# Autodesk Inventor assembly: Assembly_Mão
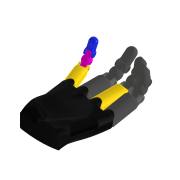
[picture p0: Inventor's stored thumbnail of the model, 180x180]
Saved by Autodesk Inventor 2020 (Build 240168000, 168)
## iProperties
Created: 2021-03-31
Part Number: Assembly_Mão
Document SubType Name: Assembly
Designer: deox
Author: deox
## Documents named in this file (17)
- C:\Users\deox\Desktop\TCC\Inventor Files\Dedo Kick\Assembly_Mão.iam
- C:\Users\deox\Desktop\TCC\Inventor Files\Dedo Kick\Base da Mão.ipt
- C:\Users\deox\Desktop\TCC\Inventor Files\Dedo Kick\Socket_Minimo.ipt
- C:\Users\deox\Desktop\TCC\Inventor Files\Dedo Kick\Cross_Minimo.ipt
- C:\Users\deox\Desktop\TCC\Inventor Files\Dedo Kick\Cross_Normal.ipt
- C:\Users\deox\Desktop\TCC\Inventor Files\Dedo Kick\Socket.ipt
- C:\Users\deox\Desktop\TCC\Inventor Files\Dedo Kick\Socket_Medio.ipt
- C:\Users\deox\Desktop\TCC\Inventor Files\Dedo Kick\Base_Minimo.ipt
- C:\Users\deox\Desktop\TCC\Inventor Files\Dedo Kick\Base.ipt
- C:\Users\deox\Desktop\TCC\Inventor Files\Dedo Kick\Middle_Minimo.ipt
- C:\Users\deox\Desktop\TCC\Inventor Files\Dedo Kick\Middle.ipt
- C:\Users\deox\Desktop\TCC\Inventor Files\Dedo Kick\ShameHider_Minimo.ipt
- C:\Users\deox\Desktop\TCC\Inventor Files\Dedo Kick\ShameHider.ipt
- C:\Users\deox\Desktop\TCC\Inventor Files\Dedo Kick\Tip_Minimo_ScaledDown.ipt
- C:\Users\deox\Desktop\TCC\Inventor Files\Dedo Kick\Tip.ipt
- C:\Users\deox\Desktop\TCC\Inventor Files\Dedo Kick\TipTip_Minimo.ipt
- C:\Users\deox\Desktop\TCC\Inventor Files\Dedo Kick\TipTip.ipt
## Components (29 placed, 16 different names)
1. Base da Mão:1 — Mate:3, Mate:4, Angle:1, Mate:7, Mate:8, Angle:2, Mate:11, Mate:12, Angle:3, Mate:15, Mate:16, Angle:4
2. Socket_Minimo:1 — Mate:1, Mate:2, Angle:1, Mate:17, Mate:18, Angle:5
3. Cross_Minimo:1 — Mate:1, Mate:2, Mate:3, Mate:4
4. Cross_Normal:1 — Mate:13, Mate:14, Mate:15, Mate:16
5. Cross_Normal:2 — Mate:9, Mate:10, Mate:11, Mate:12
6. Cross_Normal:3 — Mate:5, Mate:6, Mate:7, Mate:8
7. Socket:1 — Mate:13, Mate:14, Angle:4, Mate:23, Mate:24, Angle:8
8. Socket:2 — Mate:9, Mate:10, Angle:3, Mate:19, Mate:20, Angle:6
9. Socket_Medio:1 — Mate:5, Mate:6, Angle:2, Mate:21, Mate:22, Angle:7
10. Base_Minimo:1 — Mate:17, Mate:18, Angle:5, Mate:25, Mate:26
11. Base:1 — Mate:23, Mate:24, Angle:8, Mate:31, Mate:32
12. Base:2 — Mate:21, Mate:22, Angle:7, Mate:29, Mate:30
13. Base:3 — Mate:19, Mate:20, Angle:6, Mate:27, Mate:28
14. Middle_Minimo:1 — Mate:25, Mate:26, Mate:33, Mate:34, Mate:35, Mate:45, Mate:46
15. Middle:1 — Mate:27, Mate:28, Mate:36, Mate:37, Mate:38, Mate:47, Mate:48
16. Middle:2 — Mate:31, Mate:32, Mate:42, Mate:43, Mate:44, Mate:51, Mate:52
17. Middle:3 — Mate:29, Mate:30, Mate:39, Mate:40, Mate:41, Mate:49, Mate:50
18. ShameHider_Minimo:1 — Mate:33, Mate:34, Mate:35
19. ShameHider:1 — Mate:42, Mate:43, Mate:44
20. ShameHider:2 — Mate:39, Mate:40, Mate:41
21. ShameHider:3 — Mate:36, Mate:37, Mate:38
22. Tip_Minimo_ScaledDown:1 — Mate:45, Mate:46, Mate:53, Mate:60
23. Tip:1 — Mate:47, Mate:48, Mate:54, Mate:59
24. Tip:2 — Mate:49, Mate:50, Mate:55, Mate:58
25. Tip:3 — Mate:51, Mate:52, Mate:56, Mate:57
26. TipTip_Minimo:1 — Mate:53, Mate:60
27. TipTip:1 — Mate:54, Mate:59
28. TipTip:2 — Mate:55, Mate:58
29. TipTip:3 — Mate:56, Mate:57
## Relationships (68: Mate 60, Angle 8)
- Mate:1: Socket_Minimo:1 ↔ Cross_Minimo:1
- Mate:2: Socket_Minimo:1 ↔ Cross_Minimo:1
- Mate:3: Base da Mão:1 ↔ Cross_Minimo:1
- Mate:4: Base da Mão:1 ↔ Cross_Minimo:1
- Angle:1 (0 deg): Base da Mão:1 ↔ Socket_Minimo:1
- Mate:5: Cross_Normal:3 ↔ Socket_Medio:1
- Mate:6: Cross_Normal:3 ↔ Socket_Medio:1
- Mate:7: Base da Mão:1 ↔ Cross_Normal:3
- Mate:8: Base da Mão:1 ↔ Cross_Normal:3
- Angle:2 (0 deg): Base da Mão:1 ↔ Socket_Medio:1
- Mate:9: Cross_Normal:2 ↔ Socket:2
- Mate:10: Cross_Normal:2 ↔ Socket:2
- Mate:11: Base da Mão:1 ↔ Cross_Normal:2
- Mate:12: Base da Mão:1 ↔ Cross_Normal:2
- Angle:3 (0 deg): Base da Mão:1 ↔ Socket:2
- Mate:13: Cross_Normal:1 ↔ Socket:1
- Mate:14: Cross_Normal:1 ↔ Socket:1
- Mate:15: Base da Mão:1 ↔ Cross_Normal:1
- Mate:16: Base da Mão:1 ↔ Cross_Normal:1
- Angle:4 (0 deg): Base da Mão:1 ↔ Socket:1
- Mate:17: Socket_Minimo:1 ↔ Base_Minimo:1
- Mate:18: Socket_Minimo:1 ↔ Base_Minimo:1
- Angle:5 (0 deg): Socket_Minimo:1 ↔ Base_Minimo:1
- Mate:19: Socket:2 ↔ Base:3
- Mate:20: Socket:2 ↔ Base:3
- Angle:6 (0 deg): Socket:2 ↔ Base:3
- Mate:21: Socket_Medio:1 ↔ Base:2
- Mate:22: Socket_Medio:1 ↔ Base:2
- Angle:7 (0 deg): Socket_Medio:1 ↔ Base:2
- Mate:23: Socket:1 ↔ Base:1
- Mate:24: Socket:1 ↔ Base:1
- Angle:8 (0 deg): Socket:1 ↔ Base:1
- Mate:25: Base_Minimo:1 ↔ Middle_Minimo:1
- Mate:26: Base_Minimo:1 ↔ Middle_Minimo:1
- Mate:27: Base:3 ↔ Middle:1
- Mate:28: Base:3 ↔ Middle:1
- Mate:29: Base:2 ↔ Middle:3
- Mate:30: Base:2 ↔ Middle:3
- Mate:31: Base:1 ↔ Middle:2
- Mate:32: Base:1 ↔ Middle:2
- Mate:33: Middle_Minimo:1 ↔ ShameHider_Minimo:1
- Mate:34: Middle_Minimo:1 ↔ ShameHider_Minimo:1
- Mate:35: Middle_Minimo:1 ↔ ShameHider_Minimo:1
- Mate:36: Middle:1 ↔ ShameHider:3
- Mate:37: Middle:1 ↔ ShameHider:3
- Mate:38: Middle:1 ↔ ShameHider:3
- Mate:39: Middle:3 ↔ ShameHider:2
- Mate:40: Middle:3 ↔ ShameHider:2
- Mate:41: Middle:3 ↔ ShameHider:2
- Mate:42: Middle:2 ↔ ShameHider:1
- Mate:43: Middle:2 ↔ ShameHider:1
- Mate:44: Middle:2 ↔ ShameHider:1
- Mate:45: Middle_Minimo:1 ↔ Tip_Minimo_ScaledDown:1
- Mate:46: Middle_Minimo:1 ↔ Tip_Minimo_ScaledDown:1
- Mate:47: Middle:1 ↔ Tip:1
- Mate:48: Middle:1 ↔ Tip:1
- Mate:49: Middle:3 ↔ Tip:2
- Mate:50: Middle:3 ↔ Tip:2
- Mate:51: Middle:2 ↔ Tip:3
- Mate:52: Middle:2 ↔ Tip:3
- Mate:53: Tip_Minimo_ScaledDown:1 ↔ TipTip_Minimo:1
- Mate:54: Tip:1 ↔ TipTip:1
- Mate:55: Tip:2 ↔ TipTip:2
- Mate:56: Tip:3 ↔ TipTip:3
- Mate:57: Tip:3 ↔ TipTip:3
- Mate:58: Tip:2 ↔ TipTip:2
- Mate:59: Tip:1 ↔ TipTip:1
- Mate:60: Tip_Minimo_ScaledDown:1 ↔ TipTip_Minimo:1
